# Autodesk Inventor assembly: final_ass
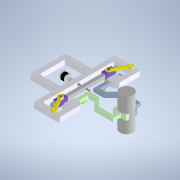
[picture p0: Inventor's stored thumbnail of the model, 180x180]
Saved by Autodesk Inventor 2021 (Build 250183000, 183)
## iProperties
Created: 2022-06-12
Part Number: final_ass
Document SubType Name: Assembly
Designer: authe
Author: authe
## Documents named in this file (11)
- C:\Users\authe\OneDrive\Desktop\Gripper7Inv\final_ass.iam
- C:\Users\authe\OneDrive\Desktop\Gripper7Inv\Frame_.ipt
- C:\Users\authe\OneDrive\Desktop\Gripper7Inv\SlderB_.ipt
- C:\Users\authe\OneDrive\Desktop\Gripper7Inv\SlderC_.ipt
- C:\Users\authe\OneDrive\Desktop\Gripper7Inv\SERVO  KH56KM2U121.iam
- C:\Users\authe\OneDrive\Desktop\Gripper7Inv\Piston_.ipt
- C:\Users\authe\OneDrive\Desktop\Gripper7Inv\SlderA_.ipt
- C:\Users\authe\OneDrive\Desktop\Gripper7Inv\Bar1_.ipt
- C:\Users\authe\OneDrive\Desktop\Gripper7Inv\Screw_.ipt
- C:\Users\authe\OneDrive\Desktop\Gripper7Inv\LAP RAP KHOP NOI MEM.iam
- C:\Users\authe\OneDrive\Desktop\Gripper7Inv\object.ipt
## Components (15 placed, 10 different names)
1. Frame_:2 — Mate:1, Mate:2, Mate:3, Mate:4, Mate:8, Mate:9, Mate:12, Mate:37, Angle:1, Mate:41
2. SlderB_:1 — Mate:1, Mate:2, Mate:16, Mate:35
3. SERVO  KH56KM2U121:1 [sub-assembly] — Mate:37, Angle:1, Mate:38, Mate:43, Mate:49
4. SlderC_:1 — Mate:3, Mate:4, Mate:19, Mate:21
5. Bar1_:1 — Mate:8, Mate:9, Mate:23
6. Bar1_:2 — Mate:12, Mate:22, Mate:28
7. Bar1_:3 — Mate:16, Mate:23, Mate:29, Mate:34, Mate:35
8. Bar1_:4 — Mate:19, Mate:21, Mate:22
9. SlderA_:1 — Mate:29, Mate:34, Mate:44, Mate:45
10. SlderA_:2 — Mate:28, Mate:47, Mate:48
11. Screw_:1 — Mate:38, Mate:40, Mate:41, Mate:42, Mate:46
12. LAP RAP KHOP NOI MEM:3 [sub-assembly] — Mate:40, Mate:42, Mate:43
13. object:1
14. Piston_:1 — Mate:44, Mate:45, Mate:46, Mate:47, Mate:48
15. LAP RAP KHOP NOI MEM:4 [sub-assembly] — Mate:49
## Relationships (29: Mate 28, Angle 1)
- Mate:1: Frame_:2 ↔ SlderB_:1
- Mate:2: Frame_:2 ↔ SlderB_:1
- Mate:3: Frame_:2 ↔ SlderC_:1
- Mate:4: Frame_:2 ↔ SlderC_:1
- Mate:8: Frame_:2 ↔ Bar1_:1
- Mate:9: Frame_:2 ↔ Bar1_:1
- Mate:12: Frame_:2 ↔ Bar1_:2
- Mate:16: SlderB_:1 ↔ Bar1_:3
- Mate:19: SlderC_:1 ↔ Bar1_:4
- Mate:21: SlderC_:1 ↔ Bar1_:4
- Mate:22: Bar1_:2 ↔ Bar1_:4
- Mate:23: Bar1_:1 ↔ Bar1_:3
- Mate:28: Bar1_:2 ↔ SlderA_:2
- Mate:29: Bar1_:3 ↔ SlderA_:1
- Mate:34: Bar1_:3 ↔ SlderA_:1
- Mate:35: SlderB_:1 ↔ Bar1_:3
- Mate:37: Frame_:2 ↔ SERVO  KH56KM2U121:1
- Angle:1 (90 deg): Frame_:2 ↔ SERVO  KH56KM2U121:1
- Mate:38: SERVO  KH56KM2U121:1 ↔ Screw_:1
- Mate:40: Screw_:1 ↔ LAP RAP KHOP NOI MEM:3
- Mate:41: Frame_:2 ↔ Screw_:1
- Mate:42: Screw_:1 ↔ LAP RAP KHOP NOI MEM:3
- Mate:43: SERVO  KH56KM2U121:1 ↔ LAP RAP KHOP NOI MEM:3
- Mate:44: SlderA_:1 ↔ Piston_:1
- Mate:45: SlderA_:1 ↔ Piston_:1
- Mate:46: Screw_:1 ↔ Piston_:1
- Mate:47: SlderA_:2 ↔ Piston_:1
- Mate:48: SlderA_:2 ↔ Piston_:1
- Mate:49: SERVO  KH56KM2U121:1 ↔ LAP RAP KHOP NOI MEM:4
